# Autodesk Inventor assembly: body
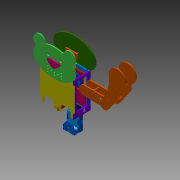
[picture p0: Inventor's stored thumbnail of the model, 180x180]
Saved by Autodesk Inventor 2013 (Build 170138000, 138)
## iProperties
Created: 2012-09-08
Part Number: body
Document SubType Name: Assembly
Designer: frankenteddy
Author: frankenteddy
## Documents named in this file (18)
- C:\Users\frankenteddy\Desktop\oshawatt1\body.iam
- C:\Users\frankenteddy\Desktop\oshawatt1\body-back.ipt
- C:\Users\frankenteddy\Desktop\oshawatt1\body-front.ipt
- C:\Users\frankenteddy\Desktop\oshawatt1\body-side.ipt
- C:\Users\frankenteddy\Desktop\oshawatt1\body-clips.ipt
- C:\Users\frankenteddy\Desktop\oshawatt1\arm-servo.ipt
- C:\Users\frankenteddy\Desktop\oshawatt1\arm-brack.iam
- C:\Users\frankenteddy\Desktop\oshawatt1\head-scotchyoke.ipt
- C:\Users\frankenteddy\Desktop\oshawatt1\head-scotchyoke-circle.ipt
- C:\Users\frankenteddy\Desktop\oshawatt1\body-scotchyoke-plate.ipt
- C:\Users\frankenteddy\Desktop\oshawatt1\body-scotchyoke-supports.ipt
- C:\Users\frankenteddy\Desktop\oshawatt1\body-clip-bottom.ipt
- C:\Users\frankenteddy\Desktop\oshawatt1\head-strut.ipt
- C:\Users\frankenteddy\Desktop\oshawatt1\head-back.ipt
- C:\Users\frankenteddy\Desktop\oshawatt1\head-front.ipt
- C:\Users\frankenteddy\Desktop\oshawatt1\head-nose.ipt
- C:\Users\frankenteddy\Desktop\oshawatt1\arm-assembled.iam
- C:\Users\frankenteddy\Desktop\oshawatt1\foot-assembled.iam
## Components (18 placed, 17 different names)
1. body-back:1 — Mate:7, Mate:8, Mate:9, Mate:10
2. body-front:1
3. body-side:1 — Mate:10
4. body-clips:1 — Mate:7, Mate:8, Mate:9
5. arm-servo:1
6. arm-brack:1 [sub-assembly]
7. head-scotchyoke:1
8. head-scotchyoke-circle:1
9. body-scotchyoke-plate:1
10. body-scotchyoke-supports:1
11. body-clip-bottom:1
12. head-strut:1
13. head-back:1
14. head-front:1
15. head-nose:1
16. arm-assembled:1 [sub-assembly]
17. foot-assembled:1 [sub-assembly]
18. foot-assembled:2 [sub-assembly]
## Relationships (4: Mate 4)
- Mate:7: body-back:1 ↔ body-clips:1
- Mate:8: body-back:1 ↔ body-clips:1
- Mate:9: body-back:1 ↔ body-clips:1
- Mate:10: body-back:1 ↔ body-side:1
